# Autodesk Inventor assembly: AA_battery_set
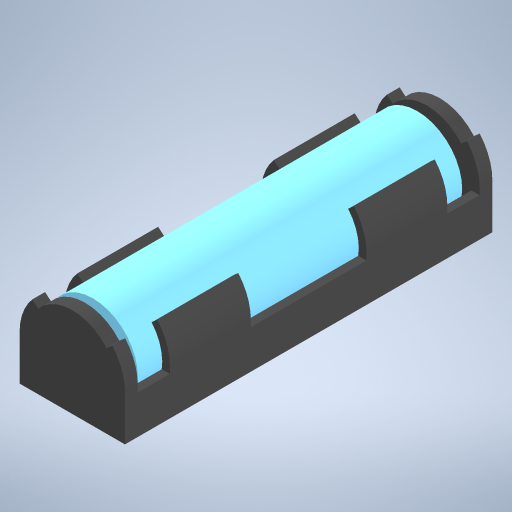
[picture p0: Inventor's stored thumbnail of the model, 512x512]
Saved by Autodesk Inventor 2024.1 (Build 281209000, 209)
## iProperties
Created: 2025-02-19
Part Number: AA_battery_set
Document SubType Name: Assembly
Designer: hibik
Author: hibik
## Documents named in this file (3)
- C:\Users\hibik\Documents\Robomech\RESCUE\ORCA\hard\std_parts\AA_battery_set.iam
- C:\Users\hibik\Documents\Robomech\RESCUE\ORCA\hard\std_parts\AA_battery_box.ipt
- C:\Users\hibik\Documents\Robomech\RESCUE\ORCA\hard\std_parts\AA_battery.ipt
## Components (2 placed, 2 different names)
1. AA_battery_box:1 — 挿入:1
2. AA_battery:1 — 挿入:1
## Relationships (1: Insert 1)
- 挿入:1 [Insert] (1.5 mm): AA_battery_box:1 ↔ AA_battery:1
